# Autodesk Inventor assembly: Motor Mount with Motor
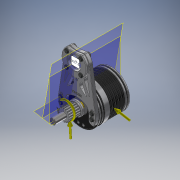
[picture p0: Inventor's stored thumbnail of the model, 180x180]
Saved by Autodesk Inventor 2019.3 (Build 233278000, 278)
## iProperties
Created: 2019-03-01
Part Number: Motor Mount with Motor
Document SubType Name: Assembly
Designer: Petar
Mass: 37.7633 g
Surface Area: 102.459 cm^2
Volume: 12.7696 cm^3
Density: 2.95729 g/cm^3
Author: Petar
## Documents named in this file (12)
- D:\OMG\E-Board\CAD\Inventor\Motor Mount with Motor.iam
- D:\OMG\E-Board\CAD\Inventor\Mechanical Components\Motor Holder v3.ipt
- D:\OMG\E-Board\CAD\Inventor\Mechanical Components\Motor Mount.ipt
- D:\OMG\E-Board\CAD\Inventor\Motor Mount\Design Accelerator\Bolted Connection1.iam
- D:\OMG\E-Board\CAD\Inventor\Motor Mount\Design Accelerator\Bolted Connection2.iam
- D:\OMG\E-Board\CAD\Inventor\Motor Mount\Design Accelerator\Bolted Connection3.iam
- D:\OMG\E-Board\CAD\Inventor\Motor Mount\Design Accelerator\Bolted Connection4.iam
- D:\OMG\E-Board\CAD\Inventor\Electric Motor\Turnigy SK8 5045.iam
- D:\OMG\E-Board\CAD\Inventor\Motor Mount with Motor\Design Accelerator\Bolted Connection1.iam
- D:\OMG\E-Board\CAD\Inventor\Motor Mount with Motor\Design Accelerator\Bolted Connection2.iam
- D:\OMG\E-Board\CAD\Inventor\Motor Mount with Motor\Design Accelerator\Bolted Connection3.iam
- D:\OMG\E-Board\CAD\Inventor\Motor Mount with Motor\Design Accelerator\Bolted Connection4.iam
## Components (11 placed, 4 different names)
1. Motor Holder v3:1 — Mate:4, Mate:5, Mate:6, Mate:8, Mate:10, Mate:12, Mate:14, Mate:15, Mate:16, Mate:17, Mate:18, Mate:20, Mate:22, Mate:24
2. Motor Mount:1 — Mate:4, Mate:5, Mate:6, Mate:7, Mate:9, Mate:11, Mate:13, Mate:26
3. Bolted Connection:1 [sub-assembly] — Mate:7, Mate:8
4. Bolted Connection:2 [sub-assembly] — Mate:9, Mate:10
5. Bolted Connection:3 [sub-assembly] — Mate:11, Mate:12
6. Bolted Connection:4 [sub-assembly] — Mate:13, Mate:14
7. Turnigy SK8 5045:1 [sub-assembly] — Mate:15, Mate:16, Mate:17, Mate:19, Mate:21, Mate:23, Mate:25, Mate:27
8. Bolted Connection:5 [sub-assembly] — Mate:18, Mate:19
9. Bolted Connection:6 [sub-assembly] — Mate:20, Mate:21
10. Bolted Connection:7 [sub-assembly] — Mate:22, Mate:23
11. Bolted Connection:8 [sub-assembly] — Mate:24, Mate:25
## Relationships (30: Mate 28, Angle 2)
- Mate:4: Motor Holder v3:1 ↔ Motor Mount:1
- Mate:5: Motor Holder v3:1 ↔ Motor Mount:1
- Mate:6: Motor Holder v3:1 ↔ Motor Mount:1
- Mate:7: Motor Mount:1 ↔ Bolted Connection:1
- Mate:8: Motor Holder v3:1 ↔ Bolted Connection:1
- Mate:9: Motor Mount:1 ↔ Bolted Connection:2
- Mate:10: Motor Holder v3:1 ↔ Bolted Connection:2
- Mate:11: Motor Mount:1 ↔ Bolted Connection:3
- Mate:12: Motor Holder v3:1 ↔ Bolted Connection:3
- Mate:13: Motor Mount:1 ↔ Bolted Connection:4
- Mate:14: Motor Holder v3:1 ↔ Bolted Connection:4
- Mate:15: Motor Holder v3:1 ↔ Turnigy SK8 5045:1
- Mate:16: Motor Holder v3:1 ↔ Turnigy SK8 5045:1
- Mate:17: Motor Holder v3:1 ↔ Turnigy SK8 5045:1
- Mate:18: Motor Holder v3:1 ↔ Bolted Connection:5
- Mate:19: Turnigy SK8 5045:1 ↔ Bolted Connection:5
- Mate:20: Motor Holder v3:1 ↔ Bolted Connection:6
- Mate:21: Turnigy SK8 5045:1 ↔ Bolted Connection:6
- Mate:22: Motor Holder v3:1 ↔ Bolted Connection:7
- Mate:23: Turnigy SK8 5045:1 ↔ Bolted Connection:7
- Mate:24: Motor Holder v3:1 ↔ Bolted Connection:8
- Mate:25: Turnigy SK8 5045:1 ↔ Bolted Connection:8
- Mate:26: Motor Mount:1
- Mate:27: Turnigy SK8 5045:1
- Mate:28
- Mate:29
- Mate:30
- Angle:1 (10 deg)
- Mate:31
- Angle:2 (90 deg)
## Named parameters: sa_0 = -1888.58, sa_1 = 4.631e-10, sa_2 = 33679.1, sa_3 = 338.445, sa_4 = 15900
note: some values were not read from the file. Shown as the stored number, unit unknown: "sa_0", "sa_1", "sa_2", "sa_3", "sa_4".
